# Autodesk Inventor assembly: Apparatus Master Assembly V1
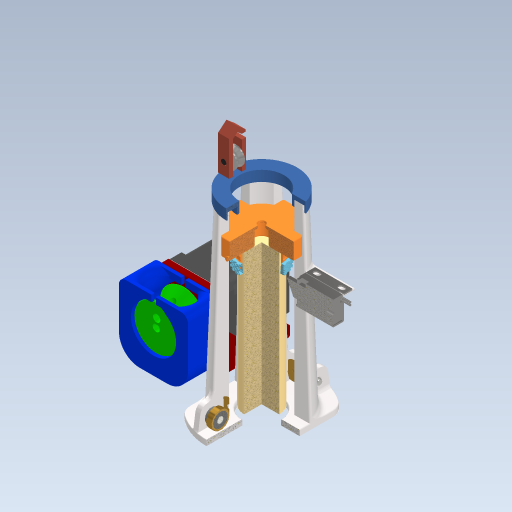
[picture p0: Inventor's stored thumbnail of the model, 512x512]
Saved by Autodesk Inventor 2023 (Build 270158000, 158)
## iProperties
Created: 2022-07-28
Part Number: Apparatus Master Assembly V1
Document SubType Name: Assembly
Designer: david
Author: david
## Documents named in this file (18)
- C:\Users\Dave\Documents\GrabCAD\Chalk Bot\Chalkbot1.0\Apparatus\V3\Apparatus Master Assembly V1.iam
- C:\Users\Dave\Documents\GrabCAD\Chalk Bot\Chalkbot1.0\Apparatus\V3\Apparatus Collet V6 CF Springs.ipt
- C:\Users\Dave\Documents\GrabCAD\Chalk Bot\Chalkbot1.0\Apparatus\V3\Spring Hubs and Shafts\1lb CF Spring Hub V1.ipt
- C:\Users\Dave\Documents\GrabCAD\Chalk Bot\Chalkbot1.0\Apparatus\V3\Cap and Cap Rope Guide\Cap Pulley Support V2 Pt2.ipt
- C:\Users\Dave\Documents\GrabCAD\Chalk Bot\Chalkbot1.0\Apparatus\V3\Cap and Cap Rope Guide\Cap Pulley Support V2 Pt1.ipt
- C:\Users\Dave\Documents\GrabCAD\Chalk Bot\Chalkbot1.0\Apparatus\V3\Cap and Cap Rope Guide\Cap V7 (Collet App).ipt
- C:\Users\Dave\Documents\GrabCAD\Chalk Bot\Chalkbot1.0\Apparatus\V3\Cap and Cap Rope Guide\Cap Pulley Support Shaft V1.ipt
- C:\Users\Dave\Documents\GrabCAD\Chalk Bot\Chalkbot1.0\Apparatus\V3\Purchased Parts\17HS19-2004S1.ipt
- C:\Users\Dave\Documents\GrabCAD\Chalk Bot\Chalkbot1.0\Apparatus\V3\Stepper Attachments\Stepper Mount V4.ipt
- C:\Users\Dave\Documents\GrabCAD\Chalk Bot\Chalkbot1.0\Apparatus\V3\Stepper Attachments\Rope Guide V5.ipt
- C:\Users\Dave\Documents\GrabCAD\Chalk Bot\Chalkbot1.0\Apparatus\V3\Stepper Attachments\Stepper Pulley V12.ipt
- C:\Users\Dave\Documents\GrabCAD\Chalk Bot\Chalkbot1.0\Apparatus\V3\Purchased Parts\LCF 025 05 031S (on hub).ipt
- C:\Users\Dave\Documents\GrabCAD\Chalk Bot\Chalkbot1.0\Apparatus\V3\Purchased Parts\Solenoid Lock.ipt
- C:\Users\Dave\Documents\GrabCAD\Chalk Bot\Chalkbot1.0\Apparatus\V3\Chalk Holder\Collet Ring V6 (4mm p).ipt
- C:\Users\Dave\Documents\GrabCAD\Chalk Bot\Chalkbot1.0\Apparatus\V3\Chalk Holder\Slider V8 (4mm pitch).ipt
- C:\Users\Dave\Documents\GrabCAD\Chalk Bot\Chalkbot1.0\Apparatus\V3\Spring Hubs and Shafts\CF Spring Shaft V1.ipt
- C:\Users\Dave\Documents\GrabCAD\Chalk Bot\Chalkbot1.0\Apparatus\V3\Purchased Parts\Chalk.ipt
- C:\Users\Dave\Documents\GrabCAD\Chalk Bot\Chalkbot1.0\Apparatus\V3\Purchased Parts\Rope Bearing Pulley.ipt
## Components (20 placed, 17 different names)
1. Apparatus Collet V6 CF Springs:1 — Insert:2, Insert:3, Mate:4, Cylindrical:1, Rotational:1, Insert:10, Insert:11
2. Solenoid Lock:1 — Mate:4
3. LCF 025 05 031S (on hub):1 — Insert:7
4. LCF 025 05 031S (on hub):2 — Insert:8
5. Chalk:1 — Insert:12
6. Rope Bearing Pulley:1 — Insert:13
7. 17HS19-2004S1:1 — Mate:5
8. Stepper Mount V4:1 — Mate:5, Slider:1
9. Rope Guide V5:1 — Slider:1, Insert:14
10. Stepper Pulley V12:1 — Insert:14
11. Cap Pulley Support Shaft V1:1 — Rigid:3
12. Cap Pulley Support V2 Pt1:1 — Rigid:2
13. Cap Pulley Support V2 Pt2:1 — Rigid:1, Rigid:3, Insert:13
14. Cap V7 (Collet App):1 — Rigid:1, Rigid:2, Rotational:1
15. 1lb CF Spring Hub V1:1 — Insert:3, Insert:8
16. 1lb CF Spring Hub V1:2 — Insert:2, Insert:7
17. CF Spring Shaft V1:1 — Insert:11
18. CF Spring Shaft V1:2 — Insert:10
19. Collet Ring V6 (4mm p):2 — Insert:9
20. Slider V8 (4mm pitch):2 — Insert:9, Cylindrical:1, Insert:12
## Relationships (18: Insert 10, WeldJoint 3, Mate 2, CylindricalJoint 1, RevoluteJoint 1, TranslationJoint 1)
- Insert:2 (1 mm): Apparatus Collet V6 CF Springs:1 ↔ 1lb CF Spring Hub V1:2
- Insert:3 (1 mm): Apparatus Collet V6 CF Springs:1 ↔ 1lb CF Spring Hub V1:1
- Insert:7 (2.5 mm): LCF 025 05 031S (on hub):1 ↔ 1lb CF Spring Hub V1:2
- Insert:8 (2.5 mm): LCF 025 05 031S (on hub):2 ↔ 1lb CF Spring Hub V1:1
- Mate:4: Apparatus Collet V6 CF Springs:1 ↔ Solenoid Lock:1
- Rigid:1 [WeldJoint]: Cap Pulley Support V2 Pt2:1 ↔ Cap V7 (Collet App):1
- Rigid:2 [WeldJoint]: Cap Pulley Support V2 Pt1:1 ↔ Cap V7 (Collet App):1
- Rigid:3 [WeldJoint]: Cap Pulley Support Shaft V1:1 ↔ Cap Pulley Support V2 Pt2:1
- Insert:9: Collet Ring V6 (4mm p):2 ↔ Slider V8 (4mm pitch):2
- Cylindrical:1: Apparatus Collet V6 CF Springs:1 ↔ Slider V8 (4mm pitch):2
- Rotational:1 [RevoluteJoint]: Apparatus Collet V6 CF Springs:1 ↔ Cap V7 (Collet App):1
- Insert:10 (-1.5 mm): Apparatus Collet V6 CF Springs:1 ↔ CF Spring Shaft V1:2
- Insert:11 (-1.5 mm): Apparatus Collet V6 CF Springs:1 ↔ CF Spring Shaft V1:1
- Insert:12: Chalk:1 ↔ Slider V8 (4mm pitch):2
- Insert:13 (0.15 mm): Rope Bearing Pulley:1 ↔ Cap Pulley Support V2 Pt2:1
- Mate:5: 17HS19-2004S1:1 ↔ Stepper Mount V4:1
- Slider:1 [TranslationJoint]: Stepper Mount V4:1 ↔ Rope Guide V5:1
- Insert:14 (2 mm): Rope Guide V5:1 ↔ Stepper Pulley V12:1
